# Autodesk Inventor assembly: bottom box with container
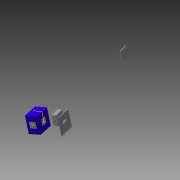
[picture p0: Inventor's stored thumbnail of the model, 180x180]
Saved by Autodesk Inventor 2015 (Build 190159000, 159)
## iProperties
Created: 2014-09-09
Part Number: bottom box with container
Document SubType Name: Assembly
Designer: ericd_000
Author: ericd_000
## Documents named in this file (12)
- C:\Users\ericd_000\Dropbox\GitHub\initial_cad\eric_cad\bottom box with container.iam
- C:\Users\ericd_000\Dropbox\GitHub\initial_cad\eric_cad\brain box bottom.ipt
- C:\Users\ericd_000\Dropbox\GitHub\initial_cad\eric_cad\bbb brick.ipt
- C:\Users\ericd_000\Dropbox\GitHub\initial_cad\eric_cad\anker20Ah.ipt
- C:\Users\ericd_000\Dropbox\GitHub\initial_cad\eric_cad\mini-itx.ipt
- C:\Users\ericd_000\Dropbox\GitHub\initial_cad\eric_cad\dlink5portswitch.ipt
- C:\Users\ericd_000\Dropbox\GitHub\initial_cad\eric_cad\stark24v10ahbattery.ipt
- C:\Users\ericd_000\Dropbox\GitHub\initial_cad\eric_cad\small24v2600mahbattery.ipt
- C:\Users\ericd_000\Dropbox\GitHub\initial_cad\eric_cad\m3.ipt
- C:\Users\ericd_000\Dropbox\GitHub\initial_cad\eric_cad\brain box top.ipt
- C:\Users\ericd_000\Dropbox\GitHub\initial_cad\eric_cad\Imported Components\M4 18mm\M4 18mm.ipt
- C:\Users\ericd_000\Dropbox\GitHub\initial_cad\eric_cad\bay con 12 mk2.iam
## Components (25 placed, 11 different names)
1. brain box bottom:1 — Mate:1, Mate:2, Mate:11, Mate:13, Mate:16, Mate:17, Mate:18, Mate:21, Mate:30, Mate:38, Mate:40, Mate:51, Cylindrical:5, Cylindrical:6, Cylindrical:9, Cylindrical:10, Mate:58, Mate:59, Mate:60, Mate:61, Cylindrical:11, Cylindrical:12, Mate:62
2. bbb brick:1 — Mate:1, Mate:2
3. anker20Ah:1 — Mate:11, Mate:12
4. anker20Ah:2 — Mate:12, Mate:13
5. mini-itx:1 — Mate:30, Mate:50
6. dlink5portswitch:1 — Mate:38
7. stark24v10ahbattery:1 — Mate:50, Mate:51
8. small24v2600mahbattery:1 — Mate:16, Mate:17
9. small24v2600mahbattery:3 — Mate:18, Mate:21
10. small24v2600mahbattery:4 — Mate:40
11. m3:1
12. m3:2
13. m3:3
14. m3:4
15. m3:5
16. m3:6
17. brain box top:1 — Cylindrical:1, Cylindrical:2, Cylindrical:3, Cylindrical:4, Mate:53, Mate:54, Mate:55, Mate:56, Cylindrical:7, Cylindrical:8, Mate:57
18. M4 18mm:1 — Cylindrical:2, Mate:55
19. M4 18mm:2 — Cylindrical:1, Mate:54, Cylindrical:6
20. M4 18mm:3 — Cylindrical:4, Mate:56, Cylindrical:5
21. M4 18mm:4 — Cylindrical:3, Mate:53
22. bay con 12 mk2:1 [sub-assembly] — Cylindrical:7, Cylindrical:8, Mate:57
23. bay con 12 mk2:2 [sub-assembly] — Mate:59, Mate:60, Mate:61
24. bay con 12 mk2:3 [sub-assembly] — Cylindrical:11, Cylindrical:12, Mate:62
25. bay con 12 mk2:4 [sub-assembly] — Cylindrical:9, Cylindrical:10, Mate:58
## Relationships (36: Mate 24, CylindricalJoint 12)
- Mate:1: brain box bottom:1 ↔ bbb brick:1
- Mate:2 (2.54 mm): brain box bottom:1 ↔ bbb brick:1
- Mate:11: brain box bottom:1 ↔ anker20Ah:1
- Mate:12 (2.54 mm): anker20Ah:1 ↔ anker20Ah:2
- Mate:13: brain box bottom:1 ↔ anker20Ah:2
- Mate:16: brain box bottom:1 ↔ small24v2600mahbattery:1
- Mate:17 (0.762 mm): brain box bottom:1 ↔ small24v2600mahbattery:1
- Mate:18: brain box bottom:1 ↔ small24v2600mahbattery:3
- Mate:21: brain box bottom:1 ↔ small24v2600mahbattery:3
- Mate:30 (38.1 mm): brain box bottom:1 ↔ mini-itx:1
- Mate:38 (2.54 mm): brain box bottom:1 ↔ dlink5portswitch:1
- Mate:40: brain box bottom:1 ↔ small24v2600mahbattery:4
- Mate:50 (2.54 mm): mini-itx:1 ↔ stark24v10ahbattery:1
- Mate:51 (52 mm): brain box bottom:1 ↔ stark24v10ahbattery:1
- Cylindrical:1: brain box top:1 ↔ M4 18mm:2
- Cylindrical:2: brain box top:1 ↔ M4 18mm:1
- Cylindrical:3: brain box top:1 ↔ M4 18mm:4
- Cylindrical:4: brain box top:1 ↔ M4 18mm:3
- Mate:53: brain box top:1 ↔ M4 18mm:4
- Mate:54: brain box top:1 ↔ M4 18mm:2
- Mate:55: brain box top:1 ↔ M4 18mm:1
- Mate:56: brain box top:1 ↔ M4 18mm:3
- Cylindrical:5: brain box bottom:1 ↔ M4 18mm:3
- Cylindrical:6: brain box bottom:1 ↔ M4 18mm:2
- Cylindrical:7: brain box top:1 ↔ bay con 12 mk2:1
- Cylindrical:8: brain box top:1 ↔ bay con 12 mk2:1
- Mate:57: brain box top:1 ↔ bay con 12 mk2:1
- Cylindrical:9: brain box bottom:1 ↔ bay con 12 mk2:4
- Cylindrical:10: brain box bottom:1 ↔ bay con 12 mk2:4
- Mate:58: brain box bottom:1 ↔ bay con 12 mk2:4
- Mate:59: brain box bottom:1 ↔ bay con 12 mk2:2
- Mate:60: brain box bottom:1 ↔ bay con 12 mk2:2
- Mate:61: brain box bottom:1 ↔ bay con 12 mk2:2
- Cylindrical:11: brain box bottom:1 ↔ bay con 12 mk2:3
- Cylindrical:12: brain box bottom:1 ↔ bay con 12 mk2:3
- Mate:62: brain box bottom:1 ↔ bay con 12 mk2:3
